# Autodesk Inventor assembly: Fish Spine
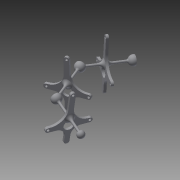
[picture p0: Inventor's stored thumbnail of the model, 180x180]
Saved by Autodesk Inventor 2015 (Build 190159000, 159)
## iProperties
Created: 2014-11-02
Part Number: Fish Spine
Document SubType Name: Assembly
Designer: Ryan
Author: Ryan
## Documents named in this file (3)
- C:\Users\Ryan\Google Drive\Documents\Berkeley\Fall 2014\EEC149\Project\FlippityFlappity\Fish Spine.iam
- C:\Users\Ryan\Google Drive\Documents\Berkeley\Fall 2014\EEC149\Project\FlippityFlappity\Fish Vertebrae.ipt
- C:\Users\Ryan\Google Drive\Documents\Berkeley\Fall 2014\EEC149\Project\FlippityFlappity\Fish Rib.ipt
## Components (6 placed, 2 different names)
1. Fish Vertebrae:1 — Mate:3, Mate:4, Mate:8
2. Fish Vertebrae:2 — Mate:5, Mate:6, Mate:7
3. Fish Vertebrae:3 — Mate:1, Mate:2, Mate:7, Mate:8
4. Fish Rib:1 — Mate:1, Mate:2
5. Fish Rib:2 — Mate:3, Mate:4
6. Fish Rib:3 — Mate:5, Mate:6
## Relationships (8: Mate 8)
- Mate:1: Fish Vertebrae:3 ↔ Fish Rib:1
- Mate:2: Fish Vertebrae:3 ↔ Fish Rib:1
- Mate:3: Fish Vertebrae:1 ↔ Fish Rib:2
- Mate:4: Fish Vertebrae:1 ↔ Fish Rib:2
- Mate:5: Fish Vertebrae:2 ↔ Fish Rib:3
- Mate:6: Fish Vertebrae:2 ↔ Fish Rib:3
- Mate:7: Fish Vertebrae:2 ↔ Fish Vertebrae:3
- Mate:8: Fish Vertebrae:1 ↔ Fish Vertebrae:3
